# Autodesk Inventor assembly: Puncher
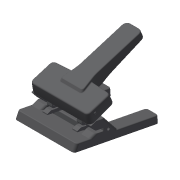
[picture p0: Inventor's stored thumbnail of the model, 180x180]
Saved by Autodesk Inventor 2022 (Build 260148000, 148)
## iProperties
Created: 2006-01-24
Part Number: Puncher
Document SubType Name: Assembly
Designer: dchu
Translation Standard: STEP AP203
File Name: C:\dom\inventor 10\Users\Train\stp\third try\Puncher.stp
Preprocessor: CATIA V5 STEP AP203
Postprocessor: Build: 211m, Release: 10 - Date: Fri 03/18/2005
Sent Units: MILLIMETERS
Uncertainty: 0.005
Author: dchu
## Documents named in this file (11)
- C:\Autodesk Inventor 2022 Advanced Assembly Modeling Practice Files\Inventor Studio - Puncher\Puncher.iam
- C:\Autodesk Inventor 2022 Advanced Assembly Modeling Practice Files\Inventor Studio - Puncher\puncher_base.ipt
- C:\Autodesk Inventor 2022 Advanced Assembly Modeling Practice Files\Inventor Studio - Puncher\Guide1.ipt
- C:\Autodesk Inventor 2022 Advanced Assembly Modeling Practice Files\Inventor Studio - Puncher\Guide2.ipt
- C:\Autodesk Inventor 2022 Advanced Assembly Modeling Practice Files\Inventor Studio - Puncher\Handle.ipt
- C:\Autodesk Inventor 2022 Advanced Assembly Modeling Practice Files\Inventor Studio - Puncher\Screw.ipt
- C:\Autodesk Inventor 2022 Advanced Assembly Modeling Practice Files\Inventor Studio - Puncher\Pin.ipt
- C:\Autodesk Inventor 2022 Advanced Assembly Modeling Practice Files\Inventor Studio - Puncher\Spring1.ipt
- C:\Autodesk Inventor 2022 Advanced Assembly Modeling Practice Files\Inventor Studio - Puncher\Screw2.ipt
- C:\Autodesk Inventor 2022 Advanced Assembly Modeling Practice Files\Inventor Studio - Puncher\Spring2.ipt
- C:\Autodesk Inventor 2022 Advanced Assembly Modeling Practice Files\Inventor Studio - Puncher\Cutter.ipt
## Components (12 placed, 7 different names)
1. Base — Mate:1, Mate:2, Mate:4, Mate:5
2. Guide:1 — Mate:1, Mate:2, Mate:3, Flush:1
3. Guide:2 — Mate:4, Mate:5, Flush:1, Mate:6
4. Cutter:1 — Mate:6, Flush:2
5. Cutter:2 — Mate:3, Flush:2
6. Spring:1
7. Spring:2
8. Screw:1
9. Screw:2
10. Handle — Mate:7
11. Pin:1
12. Pin:2 — Mate:7
## Relationships (9: Mate 7, Flush 2)
- Mate:1: Base ↔ Guide:1
- Mate:2 (5 mm): Base ↔ Guide:1
- Mate:3: Guide:1 ↔ Cutter:2
- Mate:4 (5 mm): Base ↔ Guide:2
- Mate:5: Base ↔ Guide:2
- Flush:1: Guide:1 ↔ Guide:2
- Mate:6: Guide:2 ↔ Cutter:1
- Flush:2: Cutter:1 ↔ Cutter:2
- Mate:7: Handle ↔ Pin:2
